# Autodesk Inventor assembly: VersaPlanetary 5 to 1 stage
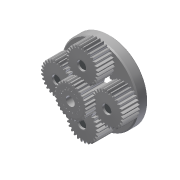
[picture p0: Inventor's stored thumbnail of the model, 180x180]
Saved by Autodesk Inventor 2013 (Build 170138000, 138)
## iProperties
Created: 2013-12-15
Part Number: VersaPlanetary 5 to 1 stage
Document SubType Name: Assembly
Designer: Nemo
Author: Nemo
## Documents named in this file (5)
- H:\Nemo\Documents\Robotics\COTS Parts\VersaPlanetary\VersaPlanetary 5 to 1 stage.iam
- H:\Nemo\Documents\Robotics\VexPro\VersaPlanetary Gearbox\Nemo VersaPlanetary Components\GR5 stage\VersaPlanetary GR5 stage plate.ipt
- H:\Nemo\Documents\Robotics\VexPro\VersaPlanetary Gearbox\Nemo VersaPlanetary Components\GR5 stage\VersaPlanetary GR5 stage sun gear.ipt
- H:\Nemo\Documents\Robotics\VexPro\VersaPlanetary Gearbox\Nemo VersaPlanetary Components\GR5 stage\VersaPlanetary GR5 stage planet axle.ipt
- H:\Nemo\Documents\Robotics\VexPro\VersaPlanetary Gearbox\Nemo VersaPlanetary Components\GR5 stage\VersaPlanetary GR5 stage planet gear.ipt
## Components (10 placed, 4 different names)
1. VersaPlanetary GR5 stage plate:1 — Insert:1, Insert:2, Mate:1, Flush:1
2. VersaPlanetary GR5 stage sun gear:1 — Mate:1, Flush:1
3. VersaPlanetary GR5 stage planet gear:1 — Insert:2
4. VersaPlanetary GR5 stage planet axle:1 — Insert:1
5. VersaPlanetary GR5 stage planet gear:2
6. VersaPlanetary GR5 stage planet axle:2
7. VersaPlanetary GR5 stage planet gear:3
8. VersaPlanetary GR5 stage planet axle:3
9. VersaPlanetary GR5 stage planet gear:4
10. VersaPlanetary GR5 stage planet axle:4
## Component patterns: (4 elements, first: VersaPlanetary GR5 stage planet gear:1 + VersaPlanetary GR5 stage planet axle:1)
## Relationships (4: Insert 2, Mate 1, Flush 1)
- Insert:1: VersaPlanetary GR5 stage plate:1 ↔ VersaPlanetary GR5 stage planet axle:1
- Insert:2: VersaPlanetary GR5 stage plate:1 ↔ VersaPlanetary GR5 stage planet gear:1
- Mate:1: VersaPlanetary GR5 stage plate:1 ↔ VersaPlanetary GR5 stage sun gear:1
- Flush:1 (13.2334 mm): VersaPlanetary GR5 stage plate:1 ↔ VersaPlanetary GR5 stage sun gear:1
